# Autodesk Inventor assembly: Part1
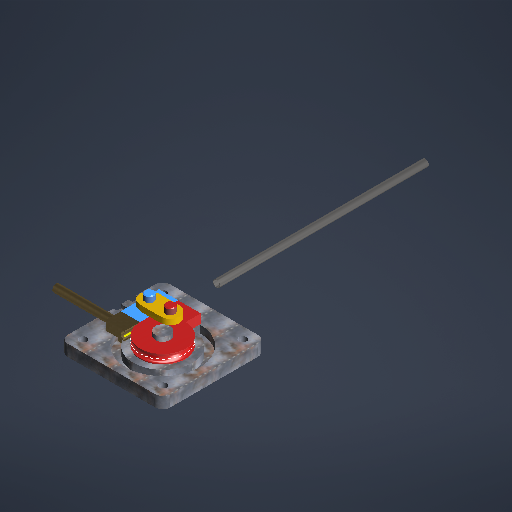
[picture p0: Inventor's stored thumbnail of the model, 512x512]
Saved by Autodesk Inventor 2026.1 (Build 301233020, 233B)
## iProperties
Created: 2025-12-25
Part Number: Part1
Document SubType Name: Assembly
Designer: kngob
Author: kngob
## Documents named in this file (7)
- C:\Users\kngob\projects\Inventor\pipe-bending-machine\bending machine assembly.iam
- C:\Users\kngob\projects\Inventor\pipe-bending-machine\parts\Bending Die.ipt
- C:\Users\kngob\projects\Inventor\pipe-bending-machine\parts\Clamp.ipt
- C:\Users\kngob\projects\Inventor\pipe-bending-machine\parts\Lever.ipt
- C:\Users\kngob\projects\Inventor\pipe-bending-machine\parts\Clip.ipt
- C:\Users\kngob\projects\Inventor\pipe-bending-machine\parts\Base.ipt
- C:\Users\kngob\projects\Inventor\pipe-bending-machine\parts\PIPE.ipt
## Components (6 placed, 6 different names)
1. Bending Die:1 — Flush:1, Flush:2, Mate:1, Mate:3
2. Clamp:1 — Flush:1, Flush:2, Mate:1, Insert:1, Flush:3, Angle:1
3. Lever:1 — Mate:2, Flush:3, Angle:1
4. Clip:1 — Insert:1
5. Base:1 — Mate:2
6. PIPE:1 — Flush:4, Mate:3, Flush:5
## Relationships (10: Flush 5, Mate 3, Insert 1, Angle 1)
- Flush:1: Bending Die:1 ↔ Clamp:1
- Flush:2: Bending Die:1 ↔ Clamp:1
- Mate:1: Bending Die:1 ↔ Clamp:1
- Insert:1: Clamp:1 ↔ Clip:1
- Mate:2: Lever:1 ↔ Base:1
- Flush:3: Clamp:1 ↔ Lever:1
- Angle:1 (0 deg): Clamp:1 ↔ Lever:1
- Flush:4 (-400 mm): PIPE:1
- Mate:3: Bending Die:1 ↔ PIPE:1
- Flush:5: PIPE:1
